# Autodesk Inventor assembly: gyroGearHeadAssembly01
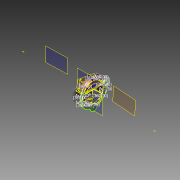
[picture p0: Inventor's stored thumbnail of the model, 180x180]
Saved by Autodesk Inventor 2013 (Build 170138000, 138)
## iProperties
Created: 2013-02-23
Part Number: gyroGearHeadAssembly01
Document SubType Name: Assembly
Designer: Nano
Author: Nano
## Documents named in this file (9)
- C:\Users\Nano\Documents\InventorByron\InventorMasterProject\gyroPhone01\gyroGearHeadAssembly01.iam
- C:\Users\Nano\Documents\InventorByron\InventorMasterProject\gyroPhone01\gear180_03.iam
- C:\Users\Nano\Documents\InventorByron\InventorMasterProject\gyroPhone01\motorWheelAssembly01.iam
- C:\Users\Nano\Documents\InventorByron\InventorMasterProject\gyroPhone01\gyroWheelCradle01.ipt
- C:\Users\Nano\Documents\InventorByron\InventorMasterProject\gyroPhone01\shortEndAxel.ipt
- C:\Users\Nano\Documents\InventorByron\InventorMasterProject\gyroPhone01\gearGuideRings.ipt
- C:\Users\Nano\Documents\InventorByron\InventorMasterProject\gyroPhone01\stepperMotorAndMount.iam
- C:\Users\Nano\Documents\InventorByron\InventorMasterProject\gyroPhone01\gyroYoke01.ipt
- C:\Users\Nano\Documents\InventorByron\InventorMasterProject\gyroPhone01\gyroYoke01_MIR.ipt
## Components (10 placed, 8 different names)
1. gear180_03:1 [sub-assembly] — Mate:6, Mate:7, Mate:8, Mate:12, Mate:13, Mate:14, Mate:15, Mate:16, Mate:17, Mate:18
2. motorWheelAssembly01:1 [sub-assembly] — Flush:1, Mate:1, Mate:2, Mate:3, Mate:4, Mate:5
3. gyroWheelCradle01:1 — Flush:1, Mate:1, Mate:2, Mate:3, Mate:4, Mate:5, Mate:6, Mate:7, Mate:8, Mate:9, Flush:2, Mate:10, Mate:11, Angle:1, Flush:20, Flush:21
4. shortEndAxel:1 — Mate:9, Flush:2
5. shortEndAxel:2 — Mate:10, Mate:11
6. gearGuideRings:1 — Mate:15, Mate:16, Mate:17, Flush:19
7. gearGuideRings:2 — Mate:12, Mate:13, Mate:14
8. stepperMotorAndMount:1 [sub-assembly] — Mate:18, Flush:19, Angle:1
9. gyroYoke01:1 — Flush:20, Flush:21
10. gyroYoke01_MIR:1
## Relationships (24: Mate 18, Flush 5, Angle 1)
- Flush:1: motorWheelAssembly01:1 ↔ gyroWheelCradle01:1
- Mate:1: motorWheelAssembly01:1 ↔ gyroWheelCradle01:1
- Mate:2 (4.7625 mm): motorWheelAssembly01:1 ↔ gyroWheelCradle01:1
- Mate:3: motorWheelAssembly01:1 ↔ gyroWheelCradle01:1
- Mate:4 (4.7625 mm): motorWheelAssembly01:1 ↔ gyroWheelCradle01:1
- Mate:5 (5.842 mm): motorWheelAssembly01:1 ↔ gyroWheelCradle01:1
- Mate:6: gear180_03:1 ↔ gyroWheelCradle01:1
- Mate:7: gear180_03:1 ↔ gyroWheelCradle01:1
- Mate:8: gear180_03:1 ↔ gyroWheelCradle01:1
- Mate:9: gyroWheelCradle01:1 ↔ shortEndAxel:1
- Flush:2: gyroWheelCradle01:1 ↔ shortEndAxel:1
- Mate:10: gyroWheelCradle01:1 ↔ shortEndAxel:2
- Mate:11: gyroWheelCradle01:1 ↔ shortEndAxel:2
- Mate:12: gear180_03:1 ↔ gearGuideRings:2
- Mate:13: gear180_03:1 ↔ gearGuideRings:2
- Mate:14: gear180_03:1 ↔ gearGuideRings:2
- Mate:15: gear180_03:1 ↔ gearGuideRings:1
- Mate:16: gear180_03:1 ↔ gearGuideRings:1
- Mate:17: gear180_03:1 ↔ gearGuideRings:1
- Mate:18: gear180_03:1 ↔ stepperMotorAndMount:1
- Flush:19: gearGuideRings:1 ↔ stepperMotorAndMount:1
- Angle:1 (0 deg): gyroWheelCradle01:1 ↔ stepperMotorAndMount:1
- Flush:20: gyroWheelCradle01:1 ↔ gyroYoke01:1
- Flush:21: gyroWheelCradle01:1 ↔ gyroYoke01:1
